# Autodesk Inventor assembly: Mano_estática
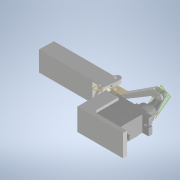
[picture p0: Inventor's stored thumbnail of the model, 180x180]
Saved by Autodesk Inventor 2020 (Build 240168000, 168)
## iProperties
Created: 2021-07-21
Part Number: Mano_estática
Document SubType Name: Assembly
Designer: chalo
Author: chalo
## Documents named in this file (6)
- C:\Users\chalo\OneDrive\Documents\GitHub\Interfaces-Biomedicas-2021\Gonzalo Palarea\Inventor\Mano_estática.iam
- C:\Users\chalo\OneDrive\Documents\GitHub\Interfaces-Biomedicas-2021\Gonzalo Palarea\Inventor\referencias\MG90_Rebuild.ipt
- C:\Users\chalo\OneDrive\Documents\GitHub\Interfaces-Biomedicas-2021\Gonzalo Palarea\Inventor\referencias\Arm01.ipt
- C:\Users\chalo\OneDrive\Documents\GitHub\Interfaces-Biomedicas-2021\Gonzalo Palarea\Inventor\Base_dedo.ipt
- C:\Users\chalo\OneDrive\Documents\GitHub\Interfaces-Biomedicas-2021\Gonzalo Palarea\Inventor\Union_dedo_base.ipt
- C:\Users\chalo\OneDrive\Documents\GitHub\Interfaces-Biomedicas-2021\Gonzalo Palarea\Inventor\Dedo_1.ipt
## Components (5 placed, 5 different names)
1. MG90_Rebuild:1 — Angle:1, Mate:1, Insert:1, Flush:2
2. Arm01:1 — Angle:1, Mate:1, Insert:1, Flush:5, Flush:6
3. Base_dedo:1 — Flush:1, Flush:2, Flush:9
4. Union_dedo_base:1 — Flush:5, Flush:6, Flush:8
5. Dedo_1:1 — Flush:7, Flush:8, Flush:9
## Relationships (10: Flush 7, Angle 1, Mate 1, Insert 1)
- Angle:1 (30 deg): MG90_Rebuild:1 ↔ Arm01:1
- Mate:1: MG90_Rebuild:1 ↔ Arm01:1
- Insert:1: MG90_Rebuild:1 ↔ Arm01:1
- Flush:1: Base_dedo:1
- Flush:2: MG90_Rebuild:1 ↔ Base_dedo:1
- Flush:5: Arm01:1 ↔ Union_dedo_base:1
- Flush:6: Arm01:1 ↔ Union_dedo_base:1
- Flush:7: Dedo_1:1
- Flush:8: Union_dedo_base:1 ↔ Dedo_1:1
- Flush:9: Base_dedo:1 ↔ Dedo_1:1
